# Autodesk Inventor assembly: Assembly1v2
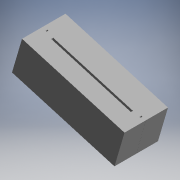
[picture p0: Inventor's stored thumbnail of the model, 180x180]
Saved by Autodesk Inventor 2017 (Build 210142000, 142)
## iProperties
Part Number: Assembly1v2
Document SubType Name: Assembly
Designer: Ole Simmering
Author: Ole Simmering
## Documents named in this file (3)
- C:\Users\Ole Simmering\Documents\GitHub\3D_modeling\Kopfhörer Ersatzteil\Assembly1v2.iam
- C:\Users\Ole Simmering\Documents\GitHub\3D_modeling\Kopfhörer Ersatzteil\Part1v2.ipt
- C:\Users\Ole Simmering\Documents\GitHub\3D_modeling\Kopfhörer Ersatzteil\Part2v2.ipt
## Components (2 placed, 2 different names)
1. Part1v2:1 — Mate:1, Mate:2, Mate:3
2. Part2v2:1 — Mate:1, Mate:2, Mate:3
## Relationships (3: Mate 3)
- Mate:1: Part1v2:1 ↔ Part2v2:1
- Mate:2: Part1v2:1 ↔ Part2v2:1
- Mate:3: Part1v2:1 ↔ Part2v2:1
